# Autodesk Inventor assembly: assembly1
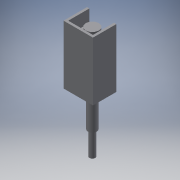
[picture p0: Inventor's stored thumbnail of the model, 180x180]
Saved by Autodesk Inventor 2018 (Build 220112000, 112)
## iProperties
Created: 2019-07-18
Part Number: assembly1
Document SubType Name: Assembly
Designer: aal_9
Author: aal_9
## Documents named in this file (8)
- C:\Users\aal_9\OneDrive\Documentos\Suiza\Courses\Tesis\CatheterLike\concepto2\assembly1.iam
- C:\Users\aal_9\OneDrive\Documentos\Suiza\Courses\Tesis\CatheterLike\concepto2\Handle.ipt
- C:\Users\aal_9\OneDrive\Documentos\Suiza\Courses\Tesis\CatheterLike\concepto2\PotSensor.ipt
- C:\Users\aal_9\OneDrive\Documentos\Suiza\Courses\Tesis\CatheterLike\concepto2\Rotation.ipt
- C:\Users\aal_9\OneDrive\Documentos\Suiza\Courses\Tesis\CatheterLike\concepto2\PotHandle.ipt
- C:\Users\aal_9\OneDrive\Documentos\Suiza\Courses\Tesis\CatheterLike\concepto2\PTA3043.ipt
- C:\Users\aal_9\OneDrive\Documentos\Suiza\Courses\Tesis\CatheterLike\concepto2\BoxBase.ipt
- C:\Users\aal_9\OneDrive\Documentos\Suiza\Courses\Tesis\CatheterLike\concepto2\Lid.ipt
## Components (7 placed, 7 different names)
1. Handle:1 — Mate:1, Flush:1, Mate:4, Mate:5, Angle:1, Angle:2, Flush:2, Mate:10, Mate:11, Mate:12, Mate:14
2. PotHandle:1 — Mate:3, Mate:4, Mate:14
3. PotSensor:1 — Mate:6, Mate:7, Mate:8, Mate:13, Flush:3
4. PTA3043:1 — Angle:1, Angle:2, Flush:2, Mate:10, Mate:11
5. Rotation:1 — Mate:1, Flush:1, Mate:3, Mate:5, Mate:6, Mate:7, Mate:8
6. BoxBase:1 — Mate:12, Mate:13, Flush:3, Mate:15, Flush:4, Mate:16
7. Lid:1 — Mate:15, Flush:4, Mate:16
## Relationships (20: Mate 14, Flush 4, Angle 2)
- Mate:1: Handle:1 ↔ Rotation:1
- Flush:1: Handle:1 ↔ Rotation:1
- Mate:3: PotHandle:1 ↔ Rotation:1
- Mate:4: Handle:1 ↔ PotHandle:1
- Mate:5 (15 mm): Handle:1 ↔ Rotation:1
- Mate:6: PotSensor:1 ↔ Rotation:1
- Mate:7: PotSensor:1 ↔ Rotation:1
- Mate:8: PotSensor:1 ↔ Rotation:1
- Angle:1 (180 deg): Handle:1 ↔ PTA3043:1
- Angle:2 (0 deg): Handle:1 ↔ PTA3043:1
- Flush:2 (-10 mm): Handle:1 ↔ PTA3043:1
- Mate:10 (4 mm): Handle:1 ↔ PTA3043:1
- Mate:11: Handle:1 ↔ PTA3043:1
- Mate:12: Handle:1 ↔ BoxBase:1
- Mate:13 (20 mm): PotSensor:1 ↔ BoxBase:1
- Flush:3 (8.5 mm): PotSensor:1 ↔ BoxBase:1
- Mate:14: Handle:1 ↔ PotHandle:1
- Mate:15: BoxBase:1 ↔ Lid:1
- Flush:4: BoxBase:1 ↔ Lid:1
- Mate:16: BoxBase:1 ↔ Lid:1
